# Autodesk Inventor assembly: Jeep
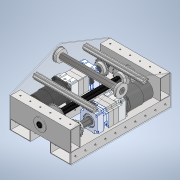
[picture p0: Inventor's stored thumbnail of the model, 180x180]
Saved by Autodesk Inventor 2020 (Build 240168000, 168)
## iProperties
Created: 2020-02-05
Part Number: Jeep
Document SubType Name: Assembly
Designer: aidan
Author: aidan
## Documents named in this file (12)
- C:\Users\aidan\Desktop\T3 Robotics\CAD\Jeep.iam
- C:\Users\aidan\Desktop\T3 Robotics\CAD\VerseFrame 6in.ipt
- C:\Users\aidan\Desktop\T3 Robotics\CAD\VerseFrame 10in.ipt
- C:\Users\aidan\Desktop\T3 Robotics\CAD\Generic and Stock\double bearing.iam
- C:\Users\aidan\Desktop\T3 Robotics\CAD\Generic and Stock\VersaPlanetary Parts\VersaPlanetary Two Stage 775 Ratchet.iam
- C:\Users\aidan\Desktop\T3 Robotics\CAD\10.25in THUNDERSHAFT.ipt
- C:\Users\aidan\Desktop\T3 Robotics\CAD\Generic and Stock\16T 22 Sprocket.ipt
- C:\Users\aidan\Desktop\T3 Robotics\CAD\Generic and Stock\22T 22 Sprocket.ipt
- C:\Users\aidan\Desktop\T3 Robotics\CAD\Jeep Plate.ipt
- C:\Users\aidan\Desktop\T3 Robotics\CAD\Bearing for THUNDER.ipt
- C:\Users\aidan\Desktop\T3 Robotics\CAD\Churro 6in.ipt
- C:\Users\aidan\Desktop\T3 Robotics\CAD\Steel Shaft for Jeep.ipt
## Components (20 placed, 11 different names)
1. VerseFrame 6in:1 — Flush:4, Flush:6, Flush:7, Flush:8, Mate:5, Mate:11
2. VerseFrame 6in:2 — Flush:2, Flush:3, Mate:1, Flush:4, Flush:5, Mate:3, Mate:4, Mate:8, Mate:10, Flush:19
3. VerseFrame 10in:1 — Flush:1, Flush:2, Flush:5, Flush:6, Flush:7, Mate:6, Flush:12, Mate:21
4. VerseFrame 10in:2 — Flush:1, Flush:3, Mate:1, Flush:8, Flush:13, Mate:22, Mate:23
5. double bearing:1 [sub-assembly] — Mate:2, Mate:5
6. double bearing:2 [sub-assembly] — Mate:2, Mate:3, Mate:4, Mate:9, Flush:10
7. VersaPlanetary Two Stage 775 Ratchet:1 [sub-assembly] — Mate:6, Mate:8, Flush:11, Mate:10, Flush:13, Mate:12, Mate:13, Mate:19
8. 10.25in THUNDERSHAFT:1 — Mate:9, Flush:10, Mate:16, Mate:17
9. VersaPlanetary Two Stage 775 Ratchet:2 [sub-assembly] — Flush:11, Mate:11, Flush:12, Mate:14, Mate:15, Mate:18
10. 16T 22 Sprocket:1 — Mate:12, Mate:13, Flush:16, Mate:19
11. 16T 22 Sprocket:2 — Mate:14, Mate:15, Flush:17, Mate:18
12. 22T 22 Sprocket:1 — Flush:14, Flush:15, Mate:16, Flush:16
13. 22T 22 Sprocket:2 — Flush:14, Flush:15, Mate:17, Flush:17
14. Jeep Plate:1 — Mate:20, Mate:21, Flush:18, Mate:24, Mate:30
15. Jeep Plate:2 — Mate:20, Mate:22, Mate:23, Flush:18, Flush:19, Mate:25, Mate:27, Mate:28, Mate:29
16. Bearing for THUNDER:1 — Mate:25, Mate:26, Mate:27, Mate:31
17. Bearing for THUNDER:2 — Mate:24, Mate:26
18. Churro 6in:1 — Flush:20, Flush:21, Mate:28
19. Churro 6in:2 — Flush:20, Flush:21, Mate:29, Mate:30
20. Steel Shaft for Jeep:1 — Mate:31
## Relationships (50: Mate 30, Flush 20)
- Flush:1: VerseFrame 10in:1 ↔ VerseFrame 10in:2
- Flush:2: VerseFrame 6in:2 ↔ VerseFrame 10in:1
- Flush:3: VerseFrame 6in:2 ↔ VerseFrame 10in:2
- Mate:1: VerseFrame 6in:2 ↔ VerseFrame 10in:2
- Flush:4: VerseFrame 6in:1 ↔ VerseFrame 6in:2
- Flush:5: VerseFrame 6in:2 ↔ VerseFrame 10in:1
- Flush:6: VerseFrame 6in:1 ↔ VerseFrame 10in:1
- Flush:7: VerseFrame 6in:1 ↔ VerseFrame 10in:1
- Flush:8: VerseFrame 6in:1 ↔ VerseFrame 10in:2
- Mate:2: double bearing:1 ↔ double bearing:2
- Mate:3: VerseFrame 6in:2 ↔ double bearing:2
- Mate:4: VerseFrame 6in:2 ↔ double bearing:2
- Mate:5: VerseFrame 6in:1 ↔ double bearing:1
- Mate:6: VerseFrame 10in:1 ↔ VersaPlanetary Two Stage 775 Ratchet:1
- Mate:8 (6.35 mm): VerseFrame 6in:2 ↔ VersaPlanetary Two Stage 775 Ratchet:1
- Mate:9: double bearing:2 ↔ 10.25in THUNDERSHAFT:1
- Flush:10 (-1.5875 mm): double bearing:2 ↔ 10.25in THUNDERSHAFT:1
- Flush:11: VersaPlanetary Two Stage 775 Ratchet:1 ↔ VersaPlanetary Two Stage 775 Ratchet:2
- Mate:10 (6.35 mm): VerseFrame 6in:2 ↔ VersaPlanetary Two Stage 775 Ratchet:1
- Mate:11 (6.35 mm): VerseFrame 6in:1 ↔ VersaPlanetary Two Stage 775 Ratchet:2
- Flush:12 (4.3942 mm): VerseFrame 10in:1 ↔ VersaPlanetary Two Stage 775 Ratchet:2
- Flush:13 (-4.3942 mm): VerseFrame 10in:2 ↔ VersaPlanetary Two Stage 775 Ratchet:1
- Mate:12: VersaPlanetary Two Stage 775 Ratchet:1 ↔ 16T 22 Sprocket:1
- Mate:13: VersaPlanetary Two Stage 775 Ratchet:1 ↔ 16T 22 Sprocket:1
- Flush:14: 22T 22 Sprocket:1 ↔ 22T 22 Sprocket:2
- Flush:15: 22T 22 Sprocket:1 ↔ 22T 22 Sprocket:2
- Mate:14: VersaPlanetary Two Stage 775 Ratchet:2 ↔ 16T 22 Sprocket:2
- Mate:15: VersaPlanetary Two Stage 775 Ratchet:2 ↔ 16T 22 Sprocket:2
- Mate:16: 10.25in THUNDERSHAFT:1 ↔ 22T 22 Sprocket:1
- Mate:17: 10.25in THUNDERSHAFT:1 ↔ 22T 22 Sprocket:2
- Flush:16: 16T 22 Sprocket:1 ↔ 22T 22 Sprocket:1
- Flush:17: 16T 22 Sprocket:2 ↔ 22T 22 Sprocket:2
- Mate:18 (25.4 mm): VersaPlanetary Two Stage 775 Ratchet:2 ↔ 16T 22 Sprocket:2
- Mate:19 (25.4 mm): VersaPlanetary Two Stage 775 Ratchet:1 ↔ 16T 22 Sprocket:1
- Mate:20: Jeep Plate:1 ↔ Jeep Plate:2
- Mate:21: VerseFrame 10in:1 ↔ Jeep Plate:1
- Mate:22: VerseFrame 10in:2 ↔ Jeep Plate:2
- Mate:23: VerseFrame 10in:2 ↔ Jeep Plate:2
- Flush:18: Jeep Plate:1 ↔ Jeep Plate:2
- Flush:19: VerseFrame 6in:2 ↔ Jeep Plate:2
- Mate:24: Jeep Plate:1 ↔ Bearing for THUNDER:2
- Mate:25: Jeep Plate:2 ↔ Bearing for THUNDER:1
- Mate:26: Bearing for THUNDER:1 ↔ Bearing for THUNDER:2
- Mate:27: Jeep Plate:2 ↔ Bearing for THUNDER:1
- Flush:20: Churro 6in:1 ↔ Churro 6in:2
- Flush:21: Churro 6in:1 ↔ Churro 6in:2
- Mate:28: Jeep Plate:2 ↔ Churro 6in:1
- Mate:29: Jeep Plate:2 ↔ Churro 6in:2
- Mate:30: Jeep Plate:1 ↔ Churro 6in:2
- Mate:31: Bearing for THUNDER:1 ↔ Steel Shaft for Jeep:1
